# Autodesk Inventor assembly: ensamble
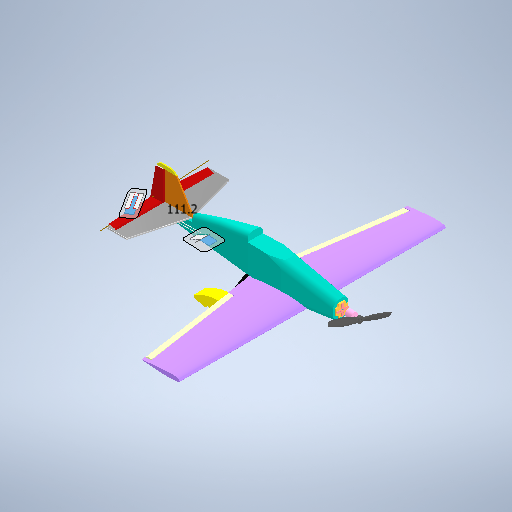
[picture p0: Inventor's stored thumbnail of the model, 512x512]
Saved by Autodesk Inventor 2025.3 (Build 293356000, 356)
## iProperties
Created: 2025-07-08
Part Number: ensamble
Document SubType Name: Assembly
Designer: jv
Author: jv
## Documents named in this file (25)
- C:\Users\steve\OneDrive\Documentos\Avion\MODELOS NUEVOS\ENSAMBLE.iam
- C:\Users\steve\OneDrive\Documentos\Avion\MODELOS NUEVOS\PARTES\BODY.ipt
- C:\Users\steve\OneDrive\Documentos\Avion\MODELOS NUEVOS\PARTES\ALA_IZQUIERDA.ipt
- C:\Users\steve\OneDrive\Documentos\Avion\MODELOS NUEVOS\PARTES\ALA_IZQUIERDA_MIR2.ipt
- C:\Users\steve\OneDrive\Documentos\Avion\MODELOS NUEVOS\ELECTRONICA\RECEPTOR.ipt
- C:\Users\steve\OneDrive\Documentos\Avion\MODELOS NUEVOS\ELECTRONICA\BATERIA.ipt
- C:\Users\steve\OneDrive\Documentos\Avion\MODELOS NUEVOS\ELECTRONICA\MOTOR.ipt
- C:\Users\steve\OneDrive\Documentos\Avion\MODELOS NUEVOS\HELICE.ipt
- C:\Users\steve\OneDrive\Documentos\Avion\MODELOS NUEVOS\WING ASSEMBLY\D.ipt
- C:\Users\steve\OneDrive\Documentos\Avion\MODELOS NUEVOS\WING ASSEMBLY\C.ipt
- C:\Users\steve\OneDrive\Documentos\Avion\MODELOS NUEVOS\WING ASSEMBLY\E.ipt
- C:\Users\steve\OneDrive\Documentos\Avion\MODELOS NUEVOS\WING ASSEMBLY\F.ipt
- C:\Users\steve\OneDrive\Documentos\Avion\MODELOS NUEVOS\PARTES\ALERO-IZQUIERDO.ipt
- C:\Users\steve\OneDrive\Documentos\Avion\MODELOS NUEVOS\PARTES\ALERO-IZQUIERDO_MIR.ipt
- C:\Users\steve\OneDrive\Documentos\Avion\MODELOS NUEVOS\WING MOUNTING\A.ipt
- C:\Users\steve\OneDrive\Documentos\Avion\MODELOS NUEVOS\AILERON LINKAGE\SERVO CAJA.iam
- C:\Users\steve\OneDrive\Documentos\Avion\MODELOS NUEVOS\MOTOR\MOTOR ENSAMBLE.iam
- C:\Users\steve\OneDrive\Documentos\Avion\MODELOS NUEVOS\HORIZONTAL STABILIZER\horizontal_stabilizer.iam
- C:\Users\steve\OneDrive\Documentos\Avion\MODELOS NUEVOS\VERTICAL_STABILIZER\vertical_stabilizer.iam
- C:\Users\steve\OneDrive\Documentos\Avion\MODELOS NUEVOS\RUDDER\Part5.ipt
- C:\Users\steve\OneDrive\Documentos\Avion\MODELOS NUEVOS\RUDDER\G.ipt
- C:\Users\steve\OneDrive\Documentos\Avion\MODELOS NUEVOS\RUDDER\mini_vara.ipt
- C:\Users\steve\OneDrive\Documentos\Avion\MODELOS NUEVOS\RUDDER\big_vara.ipt
- C:\Users\steve\OneDrive\Documentos\Avion\Servo Motor MG996R 3D Model\Servo Motor MG996R 3D Model\Servo Motor MG996R 3D Model.ipt
- C:\Users\steve\OneDrive\Documentos\Avion\MODELOS NUEVOS\Main Gear\MainGear.iam
## Components (36 placed, 24 different names)
1. BODY:1 — Angle:1, Mate:3, Mate:4, Mate:5, Flush:1, Mate:7, Mate:32, Mate:33, Mate:40, Angle:5, Mate:41, Mate:42, Angle:6, Mate:46, Mate:47, Mate:48, Mate:49, Mate:58, Mate:63
2. ALA_IZQUIERDA:1 — Mate:1, Mate:2, Angle:1, Angle:4, Mate:33, Mate:34, Mate:38, Angle:7, Mate:45
3. ALA_IZQUIERDA_MIR2:1 — Mate:1, Mate:2, Mate:12, Angle:3, Mate:16, Mate:18, Mate:21, Mate:22, Mate:24, Mate:25, Mate:26, Mate:27, Angle:4, Mate:36, Mate:37, Mate:44
4. RECEPTOR:1 — Mate:4
5. BATERIA:1 — Mate:3
6. MOTOR:1 — Mate:5, Insert:1, Mate:7
7. HELICE:1 — Insert:1
8. D:1 — Mate:16, Mate:18, Mate:19, Mate:23, Mate:24, Mate:29, Mate:30
9. C:1 — Mate:12, Angle:3, Mate:13, Mate:14, Mate:21, Mate:22, Mate:32
10. C:2 — Mate:13, Mate:14, Mate:43
11. D:2 — Mate:19, Mate:23, Mate:31
12. E:1 — Mate:25, Mate:26, Mate:27
13. F:1 — Mate:29, Mate:30, Mate:31
14. ALERO-IZQUIERDO:1 — Mate:34, Mate:38
15. ALERO-IZQUIERDO_MIR:1 — Mate:36, Mate:37
16. A:1 — Mate:40, Angle:5, Mate:41, Mate:42
17. SERVO CAJA:1 [sub-assembly] — Angle:6, Mate:43, Angle:7, Mate:44, Mate:45
18. MOTOR ENSAMBLE:1 [sub-assembly] — Mate:46, Mate:47
19. horizontal_stabilizer:1 [sub-assembly] — Mate:48, Mate:50, Mate:52, Mate:54, Mate:55, Mate:56, Mate:59, Mate:60, Mate:61
20. vertical_stabilizer:1 [sub-assembly] — Mate:49, Mate:50, Mate:53
21. Part5:1 — Mate:52, Mate:60, Mate:61, Rotational:2, Insert:11
22. Part5:2 — Mate:53, Rotational:1, Insert:9
23. Part5:3 — Mate:54, Mate:55, Insert:4
24. G:1 — Insert:6, Rotational:2, Insert:11
25. G:2 — Rotational:1, Insert:9, Insert:10
26. G:3 — Insert:4, Insert:5
27. mini_vara:1 — Insert:6, Insert:12
28. mini_vara:2 — Insert:10, Mate:62
29. mini_vara:3 — Insert:5, Insert:8
30. big_vara:1 — Insert:8
31. big_vara:2 — Mate:62
32. big_vara:3 — Insert:12
33. Servo Motor MG996R 3D Model:1
34. Servo Motor MG996R 3D Model:2
35. Servo Motor MG996R 3D Model:3
36. MainGear:1 [sub-assembly] — Mate:63
## Relationships (68: Mate 50, Insert 9, Angle 6, RevoluteJoint 2, Flush 1)
- Mate:1 (6 mm): ALA_IZQUIERDA:1 ↔ ALA_IZQUIERDA_MIR2:1
- Mate:2: ALA_IZQUIERDA:1 ↔ ALA_IZQUIERDA_MIR2:1
- Angle:1 (90 deg): BODY:1 ↔ ALA_IZQUIERDA:1
- Mate:3: BODY:1 ↔ BATERIA:1
- Mate:4: BODY:1 ↔ RECEPTOR:1
- Mate:5: BODY:1 ↔ MOTOR:1
- Flush:1: BODY:1
- Insert:1: MOTOR:1 ↔ HELICE:1
- Mate:7: BODY:1 ↔ MOTOR:1
- Mate:12: ALA_IZQUIERDA_MIR2:1 ↔ C:1
- Angle:3 (-90 deg): ALA_IZQUIERDA_MIR2:1 ↔ C:1
- Mate:13: C:1 ↔ C:2
- Mate:14: C:1 ↔ C:2
- Mate:16: ALA_IZQUIERDA_MIR2:1 ↔ D:1
- Mate:18: ALA_IZQUIERDA_MIR2:1 ↔ D:1
- Mate:19: D:1 ↔ D:2
- Mate:21: ALA_IZQUIERDA_MIR2:1 ↔ C:1
- Mate:22: ALA_IZQUIERDA_MIR2:1 ↔ C:1
- Mate:23: D:1 ↔ D:2
- Mate:24: ALA_IZQUIERDA_MIR2:1 ↔ D:1
- Mate:25: ALA_IZQUIERDA_MIR2:1 ↔ E:1
- Mate:26: ALA_IZQUIERDA_MIR2:1 ↔ E:1
- Mate:27: ALA_IZQUIERDA_MIR2:1 ↔ E:1
- Mate:29 (3 mm): D:1 ↔ F:1
- Mate:30 (4 mm): D:1 ↔ F:1
- Mate:31: D:2 ↔ F:1
- Angle:4 (0 deg): ALA_IZQUIERDA:1 ↔ ALA_IZQUIERDA_MIR2:1
- Mate:32: BODY:1 ↔ C:1
- Mate:33 (-3 mm): BODY:1 ↔ ALA_IZQUIERDA:1
- Mate:34: ALA_IZQUIERDA:1 ↔ ALERO-IZQUIERDO:1
- Mate:36: ALA_IZQUIERDA_MIR2:1 ↔ ALERO-IZQUIERDO_MIR:1
- Mate:37 (1 mm): ALA_IZQUIERDA_MIR2:1 ↔ ALERO-IZQUIERDO_MIR:1
- Mate:38 (1 mm): ALA_IZQUIERDA:1 ↔ ALERO-IZQUIERDO:1
- Mate:40: BODY:1 ↔ A:1
- Angle:5 (-80 deg): BODY:1 ↔ A:1
- Mate:41 (15 mm): BODY:1 ↔ A:1
- Mate:42: BODY:1 ↔ A:1
- Angle:6 (0 deg): BODY:1 ↔ SERVO CAJA:1
- Mate:43: C:2 ↔ SERVO CAJA:1
- Angle:7 (175 deg): ALA_IZQUIERDA:1 ↔ SERVO CAJA:1
- Mate:44: ALA_IZQUIERDA_MIR2:1 ↔ SERVO CAJA:1
- Mate:45 (-55 mm): ALA_IZQUIERDA:1 ↔ SERVO CAJA:1
- Mate:46: BODY:1 ↔ MOTOR ENSAMBLE:1
- Mate:47: BODY:1 ↔ MOTOR ENSAMBLE:1
- Mate:48: BODY:1 ↔ horizontal_stabilizer:1
- Mate:49: BODY:1 ↔ vertical_stabilizer:1
- Mate:50: horizontal_stabilizer:1 ↔ vertical_stabilizer:1
- Mate:52: horizontal_stabilizer:1 ↔ Part5:1
- Mate:53: vertical_stabilizer:1 ↔ Part5:2
- Mate:54: horizontal_stabilizer:1 ↔ Part5:3
- Mate:55: horizontal_stabilizer:1 ↔ Part5:3
- Insert:4: Part5:3 ↔ G:3
- Insert:5: G:3 ↔ mini_vara:3
- Insert:6: G:1 ↔ mini_vara:1
- Mate:56: horizontal_stabilizer:1
- Mate:58: BODY:1
- Mate:59: horizontal_stabilizer:1
- Mate:60: horizontal_stabilizer:1 ↔ Part5:1
- Mate:61: horizontal_stabilizer:1 ↔ Part5:1
- Rotational:1 [RevoluteJoint]: Part5:2 ↔ G:2
- Rotational:2 [RevoluteJoint]: Part5:1 ↔ G:1
- Insert:8: mini_vara:3 ↔ big_vara:1
- Insert:9: Part5:2 ↔ G:2
- Insert:10: G:2 ↔ mini_vara:2
- Mate:62: mini_vara:2 ↔ big_vara:2
- Insert:11: Part5:1 ↔ G:1
- Insert:12: mini_vara:1 ↔ big_vara:3
- Mate:63: BODY:1 ↔ MainGear:1
